# Autodesk Inventor assembly: Shooter
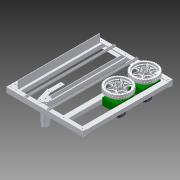
[picture p0: Inventor's stored thumbnail of the model, 180x180]
Saved by Autodesk Inventor 2013 (Build 170138000, 138)
## iProperties
Created: 2013-01-27
Part Number: Shooter
Document SubType Name: Assembly
Designer: Naphat
Author: Naphat
## Documents named in this file (11)
- C:\Users\carneeki\Desktop\Kiwi Robot\Shooter\Shooter.iam
- C:\Users\carneeki\Desktop\Kiwi Robot\Imported Components\Wheels\Basic Wheel\Shooter Basic Design.iam
- C:\Users\carneeki\Desktop\Kiwi Robot\Shooter\Shooter Pressure Channel.ipt
- C:\Users\carneeki\Desktop\Kiwi Robot\Shooter\Low Friction Frisbee Track.ipt
- C:\Users\carneeki\Desktop\Kiwi Robot\Shooter\Firing Pin\Firing Pin.iam
- C:\Users\carneeki\Desktop\Kiwi Robot\Shooter\Shooter Frame - Rear.ipt
- C:\Users\carneeki\Desktop\Kiwi Robot\Shooter\Shooter Frame - Left.ipt
- C:\Users\carneeki\Desktop\Kiwi Robot\Shooter\Shooter Frame - Right.ipt
- C:\Users\carneeki\Desktop\Kiwi Robot\Shooter\Shooter Frame - Front.ipt
- C:\Users\carneeki\Desktop\Kiwi Robot\Shooter\Shooter Frame - CIM Mount.ipt
- C:\Users\carneeki\Desktop\Kiwi Robot\Shooter\Shooter Frame - Firing Pin Mount.ipt
## Components (13 placed, 11 different names)
1. Pressure Channel — Mate:212, Mate:213, Flush:4
2. Low Friction Frisbee Track:1 — Mate:219, Insert:13
3. Low Friction Frisbee Track:2 — Mate:217, Mate:218, Insert:14, Insert:15
4. Firing Pin:1 [sub-assembly] — Mate:226, Mate:227
5. Wheel Assy:Rear [sub-assembly] — Flush:3, Insert:7, Insert:8
6. Wheel Assy:Front [sub-assembly] — Flush:3, Insert:9, Insert:10
7. Shooter Frame - Firing Pin Mount:1 — Mate:223, Mate:224, Insert:11, Insert:12, Mate:226, Mate:227
8. Shooter Frame - Rear:1 — Insert:2, Insert:4, Insert:6, Mate:213, Mate:217, Mate:218, Mate:219, Insert:11, Insert:13, Insert:14
9. Shooter Frame - Front:1 — Insert:1, Insert:3, Insert:5, Mate:214, Mate:215, Mate:223, Mate:224, Insert:12, Insert:15
10. Shooter Frame - Right:1 — Insert:1, Insert:2, Insert:7, Insert:8, Insert:9, Insert:10
11. Shooter Frame - CIM Mount:1 — Insert:3, Insert:4
12. Shooter Frame - Left:1 — Insert:5, Insert:6, Mate:212, Flush:4, Mate:216
13. Shooter Frame - Left:2 — Mate:214, Mate:215, Mate:216
## Relationships (29: Insert 15, Mate 12, Flush 2)
- Flush:3: Wheel Assy:Rear ↔ Wheel Assy:Front
- Insert:1: Shooter Frame - Front:1 ↔ Shooter Frame - Right:1
- Insert:2: Shooter Frame - Rear:1 ↔ Shooter Frame - Right:1
- Insert:3: Shooter Frame - Front:1 ↔ Shooter Frame - CIM Mount:1
- Insert:4: Shooter Frame - Rear:1 ↔ Shooter Frame - CIM Mount:1
- Insert:5: Shooter Frame - Front:1 ↔ Shooter Frame - Left:1
- Insert:6: Shooter Frame - Rear:1 ↔ Shooter Frame - Left:1
- Mate:212: Pressure Channel ↔ Shooter Frame - Left:1
- Mate:213: Pressure Channel ↔ Shooter Frame - Rear:1
- Flush:4: Pressure Channel ↔ Shooter Frame - Left:1
- Mate:214: Shooter Frame - Front:1 ↔ Shooter Frame - Left:2
- Mate:215: Shooter Frame - Front:1 ↔ Shooter Frame - Left:2
- Mate:216: Shooter Frame - Left:1 ↔ Shooter Frame - Left:2
- Mate:217: Low Friction Frisbee Track:2 ↔ Shooter Frame - Rear:1
- Mate:218: Low Friction Frisbee Track:2 ↔ Shooter Frame - Rear:1
- Mate:219: Low Friction Frisbee Track:1 ↔ Shooter Frame - Rear:1
- Insert:7: Wheel Assy:Rear ↔ Shooter Frame - Right:1
- Insert:8: Wheel Assy:Rear ↔ Shooter Frame - Right:1
- Insert:9: Wheel Assy:Front ↔ Shooter Frame - Right:1
- Insert:10: Wheel Assy:Front ↔ Shooter Frame - Right:1
- Mate:223: Shooter Frame - Firing Pin Mount:1 ↔ Shooter Frame - Front:1
- Mate:224: Shooter Frame - Firing Pin Mount:1 ↔ Shooter Frame - Front:1
- Insert:11: Shooter Frame - Firing Pin Mount:1 ↔ Shooter Frame - Rear:1
- Insert:12: Shooter Frame - Firing Pin Mount:1 ↔ Shooter Frame - Front:1
- Mate:226: Firing Pin:1 ↔ Shooter Frame - Firing Pin Mount:1
- Mate:227: Firing Pin:1 ↔ Shooter Frame - Firing Pin Mount:1
- Insert:13: Low Friction Frisbee Track:1 ↔ Shooter Frame - Rear:1
- Insert:14: Low Friction Frisbee Track:2 ↔ Shooter Frame - Rear:1
- Insert:15: Low Friction Frisbee Track:2 ↔ Shooter Frame - Front:1
